# Autodesk Inventor assembly: Revised Gearbox #1 Assembly
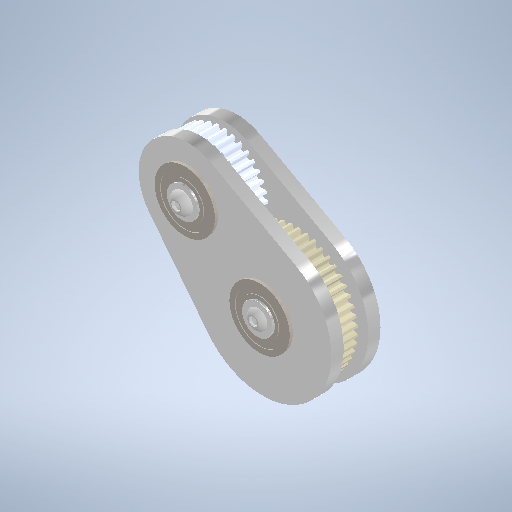
[picture p0: Inventor's stored thumbnail of the model, 512x512]
Saved by Autodesk Inventor 2025.1 (Build 291241020, 241B)
## iProperties
Created: 2024-09-16
Part Number: Revised Gearbox #1 Assembly
Document SubType Name: Assembly
Designer: xmand
Author: xmand
## Documents named in this file (8)
- C:\Users\xmand\OneDrive\Documents\GitHub\1622-2024-Assignments\Xavier Daza\Gearbox #1\Revised Gearbox #1 Assembly.iam
- C:\Users\xmand\OneDrive\Documents\GitHub\1622-2024-Assignments\Xavier Daza\Gearbox #1\Revised Gearbox Plate #1.ipt
- C:\Users\xmand\Downloads\WCP-0783\WCP-0783\WCP-0783.ipt
- C:\Users\xmand\Downloads\WCP-0709\WCP-0709\WCP-0709.ipt
- C:\Users\xmand\OneDrive\Documents\GitHub\1622-2024-Assignments\Xavier Daza\Gearbox #1\WCP-0188 (1).ipt
- C:\Users\xmand\OneDrive\Documents\GitHub\1622-2024-Assignments\Xavier Daza\Gearbox #1\1.123 hex shaft 0.25-20 0.5.ipt
- C:\Users\xmand\OneDrive\Documents\GitHub\1622-2024-Assignments\Xavier Daza\Gearbox #1\92949A535_18-8 Stainless Steel Button Head Hex Drive Screw.ipt
- C:\Users\xmand\OneDrive\Documents\GitHub\1622-2024-Assignments\Xavier Daza\Gearbox #1\90107A029_316 Stainless Steel Washer.ipt
## Components (18 placed, 7 different names)
1. Revised Gearbox Plate #1:1 — Mate:2, Mate:3, Mate:4, Mate:6, Insert:1, Insert:2
2. Revised Gearbox Plate #1:2 — Mate:2, Mate:3, Mate:5, Mate:7, Insert:3, Insert:4
3. WCP-0783:1 — Mate:5, Insert:4, Mate:9, Angle:2, Mate:15
4. WCP-0783:2 — Insert:1, Mate:10, Mate:11, Angle:3, Mate:14
5. WCP-0783:3 — Mate:7, Insert:3, Mate:8
6. WCP-0783:4 — Insert:2, Angle:1, Angle:5
7. WCP-0709:1 — Mate:4, Tangent:1, Mate:9, Angle:1, Angle:2
8. WCP-0188 (1):1 — Mate:6, Tangent:1, Mate:8, Mate:10, Mate:11, Angle:3
9. 1.123 hex shaft 0.25-20 0.5:1 — Mate:14, Mate:16, Mate:17, Insert:7, Mate:20, Mate:21, Insert:9
10. 1.123 hex shaft 0.25-20 0.5:2 — Mate:15, Angle:5, Insert:5, Mate:18, Mate:19, Insert:8
11. 92949A535_18-8 Stainless Steel Button Head Hex Drive Screw:1 — Insert:9
12. 92949A535_18-8 Stainless Steel Button Head Hex Drive Screw:2 — Insert:6
13. 92949A535_18-8 Stainless Steel Button Head Hex Drive Screw:3 — Insert:7
14. 92949A535_18-8 Stainless Steel Button Head Hex Drive Screw:4 — Insert:8
15. 90107A029_316 Stainless Steel Washer:1 — Insert:5, Insert:6
16. 90107A029_316 Stainless Steel Washer:2 — Mate:18, Mate:19
17. 90107A029_316 Stainless Steel Washer:3 — Mate:20, Mate:21
18. 90107A029_316 Stainless Steel Washer:4 — Mate:16, Mate:17
## Relationships (32: Mate 18, Insert 9, Angle 4, Tangent 1)
- Mate:2: Revised Gearbox Plate #1:1 ↔ Revised Gearbox Plate #1:2
- Mate:3: Revised Gearbox Plate #1:1 ↔ Revised Gearbox Plate #1:2
- Mate:4: Revised Gearbox Plate #1:1 ↔ WCP-0709:1
- Mate:5: Revised Gearbox Plate #1:2 ↔ WCP-0783:1
- Mate:6: Revised Gearbox Plate #1:1 ↔ WCP-0188 (1):1
- Mate:7: Revised Gearbox Plate #1:2 ↔ WCP-0783:3
- Insert:1: Revised Gearbox Plate #1:1 ↔ WCP-0783:2
- Insert:2: Revised Gearbox Plate #1:1 ↔ WCP-0783:4
- Tangent:1: WCP-0709:1 ↔ WCP-0188 (1):1
- Insert:3: Revised Gearbox Plate #1:2 ↔ WCP-0783:3
- Insert:4: Revised Gearbox Plate #1:2 ↔ WCP-0783:1
- Mate:8: WCP-0783:3 ↔ WCP-0188 (1):1
- Mate:9: WCP-0783:1 ↔ WCP-0709:1
- Mate:10: WCP-0783:2 ↔ WCP-0188 (1):1
- Mate:11: WCP-0783:2 ↔ WCP-0188 (1):1
- Angle:1 (0 deg): WCP-0783:4 ↔ WCP-0709:1
- Angle:2 (0 deg): WCP-0783:1 ↔ WCP-0709:1
- Angle:3 (0 deg): WCP-0783:2 ↔ WCP-0188 (1):1
- Mate:14: WCP-0783:2 ↔ 1.123 hex shaft 0.25-20 0.5:1
- Mate:15: WCP-0783:1 ↔ 1.123 hex shaft 0.25-20 0.5:2
- Angle:5 (0 deg): WCP-0783:4 ↔ 1.123 hex shaft 0.25-20 0.5:2
- Insert:5: 1.123 hex shaft 0.25-20 0.5:2 ↔ 90107A029_316 Stainless Steel Washer:1
- Insert:6: 92949A535_18-8 Stainless Steel Button Head Hex Drive Screw:2 ↔ 90107A029_316 Stainless Steel Washer:1
- Mate:16: 1.123 hex shaft 0.25-20 0.5:1 ↔ 90107A029_316 Stainless Steel Washer:4
- Mate:17: 1.123 hex shaft 0.25-20 0.5:1 ↔ 90107A029_316 Stainless Steel Washer:4
- Insert:7: 1.123 hex shaft 0.25-20 0.5:1 ↔ 92949A535_18-8 Stainless Steel Button Head Hex Drive Screw:3
- Mate:18: 1.123 hex shaft 0.25-20 0.5:2 ↔ 90107A029_316 Stainless Steel Washer:2
- Mate:19: 1.123 hex shaft 0.25-20 0.5:2 ↔ 90107A029_316 Stainless Steel Washer:2
- Insert:8: 1.123 hex shaft 0.25-20 0.5:2 ↔ 92949A535_18-8 Stainless Steel Button Head Hex Drive Screw:4
- Mate:20: 1.123 hex shaft 0.25-20 0.5:1 ↔ 90107A029_316 Stainless Steel Washer:3
- Mate:21: 1.123 hex shaft 0.25-20 0.5:1 ↔ 90107A029_316 Stainless Steel Washer:3
- Insert:9: 1.123 hex shaft 0.25-20 0.5:1 ↔ 92949A535_18-8 Stainless Steel Button Head Hex Drive Screw:1
